# Autodesk Inventor assembly: bumper_MIR
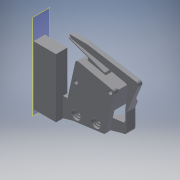
[picture p0: Inventor's stored thumbnail of the model, 180x180]
Saved by Autodesk Inventor 2016 (Build 200138000, 138)
## iProperties
Created: 2016-02-16
Part Number: bumper_MIR
Document SubType Name: Assembly
Designer: jforce
Author: jforce
## Documents named in this file (4)
- C:\Users\jforce\Dropbox\gmu\ece590 (Selective Sync Conflict)\models3\bumper_MIR.iam
- C:\Users\jforce\Dropbox\gmu\ece590 (Selective Sync Conflict)\models3\bumper_plate_MIR.ipt
- C:\Users\jforce\Dropbox\gmu\ece590 (Selective Sync Conflict)\models3\switch_MIR.ipt
- C:\Users\jforce\Dropbox\gmu\ece590 (Selective Sync Conflict)\models3\bump_switch_mount_MIR.ipt
## Components (3 placed, 3 different names)
1. bumper_plate_MIR:1
2. switch_MIR:1 — Mate:1, Flush:1
3. bump_switch_mount_MIR:1 — Mate:1, Flush:1
## Relationships (2: Mate 1, Flush 1)
- Mate:1: switch_MIR:1 ↔ bump_switch_mount_MIR:1
- Flush:1: switch_MIR:1 ↔ bump_switch_mount_MIR:1
